# Autodesk Inventor assembly: McCrea_assembly_walle
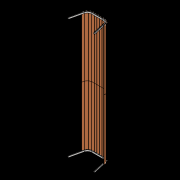
[picture p0: Inventor's stored thumbnail of the model, 180x180]
Saved by Autodesk Inventor 2021 (Build 250183000, 183)
## iProperties
Created: 2022-01-17
Part Number: McCrea_assembly_walle
Document SubType Name: Assembly
Designer: student
Author: student
## Documents named in this file (6)
- E:\Škola\teg\wall-e\matus\bench\McCrea_assembly_walle.iam
- E:\Škola\teg\wall-e\matus\bench\McCrea_doska_walle.ipt
- E:\Škola\teg\wall-e\matus\bench\McCrea_noha_walle.ipt
- E:\Škola\teg\wall-e\matus\bench\McCrea_DoskaPath_walle.ipt
- E:\Škola\teg\wall-e\matus\bench\McCrea_noha_walle_MIR.ipt
- E:\Škola\teg\wall-e\matus\bench\McCrea_doska_walle_MIR.ipt
## Components (25 placed, 5 different names)
1. McCrea_noha_walle:1 — Flush:1, Flush:2, Mate:2
2. McCrea_DoskaPath_walle:1 — Flush:1, Flush:2, Mate:1
3. McCrea_noha_walle_MIR:1
4. McCrea_doska_walle_MIR:1
5. McCrea_doska_walle_MIR:2
6. McCrea_doska_walle_MIR:3
7. McCrea_doska_walle_MIR:4
8. McCrea_doska_walle_MIR:5
9. McCrea_doska_walle_MIR:6
10. McCrea_doska_walle_MIR:7
11. McCrea_doska_walle_MIR:8
12. McCrea_doska_walle_MIR:9
13. McCrea_doska_walle_MIR:10
14. McCrea_doska_walle_MIR:11
15. McCrea_doska_walle:1 — Mate:1, Mate:2
16. McCrea_doska_walle:2
17. McCrea_doska_walle:3
18. McCrea_doska_walle:4
19. McCrea_doska_walle:5 — Flush:3
20. McCrea_doska_walle:6
21. McCrea_doska_walle:7
22. McCrea_doska_walle:8
23. McCrea_doska_walle:9
24. McCrea_doska_walle:10
25. McCrea_doska_walle:11
## Component patterns: (11 elements, first: McCrea_doska_walle:1)
## Relationships (5: Flush 3, Mate 2)
- Flush:1: McCrea_noha_walle:1 ↔ McCrea_DoskaPath_walle:1
- Flush:2: McCrea_noha_walle:1 ↔ McCrea_DoskaPath_walle:1
- Mate:1: McCrea_DoskaPath_walle:1 ↔ McCrea_doska_walle:1
- Mate:2: McCrea_noha_walle:1 ↔ McCrea_doska_walle:1
- Flush:3: McCrea_doska_walle:5
